# Autodesk Inventor assembly: Montiert
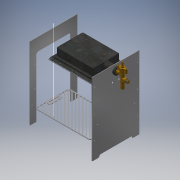
[picture p0: Inventor's stored thumbnail of the model, 180x180]
Saved by Autodesk Inventor 2018 (Build 220112000, 112)
## iProperties
Created: 2017-11-12
Part Number: Montiert
Material: Generisch
Document SubType Name: Assembly
Mass: 12109.4 g
Surface Area: 4943.53 cm^2
Volume: 1535.77 cm^3
Density: 7.8849 g/cm^3
## Documents named in this file (18)
- C:\git\RoKu-ProjectX01\Konstruktion\Montiert.iam
- C:\git\RoKu-ProjectX01\Konstruktion\Brenner.ipt
- C:\git\RoKu-ProjectX01\Konstruktion\BrennerHalter.ipt
- C:\git\RoKu-ProjectX01\Konstruktion\Gegenhalter.ipt
- C:\Users\kuckal\Documents\Inventor\Content Center Files\R2018\de-DE\ISO 7380-1\ISO 7380-1 - M4 x 6.ipt
- C:\Users\kuckal\Documents\Inventor\Content Center Files\R2018\de-DE\ISO 7380-1\ISO 7380-1 - M4 x 8.ipt
- C:\Users\kuckal\Documents\Inventor\Content Center Files\R2018\de-DE\ISO 4036(1)\ISO 4036 - M4(1).ipt
- C:\git\RoKu-ProjectX01\Konstruktion\Front.ipt
- C:\git\RoKu-ProjectX01\Konstruktion\MutterMitUScheibe.ipt
- C:\git\RoKu-ProjectX01\Konstruktion\SeiteRechts.ipt
- C:\git\RoKu-ProjectX01\Konstruktion\SeiteLinks.ipt
- C:\git\RoKu-ProjectX01\Konstruktion\Deckel.ipt
- C:\git\RoKu-ProjectX01\Konstruktion\Boden.ipt
- C:\git\RoKu-ProjectX01\Konstruktion\Back.ipt
- C:\git\RoKu-ProjectX01\Konstruktion\Gasanschluss.ipt
- C:\Users\kuckal\Documents\Inventor\Content Center Files\R2018\de-DE\DIN EN 24 036(2)\DIN EN 24 036 - M4.ipt
- C:\git\RoKu-ProjectX01\Konstruktion\EinschubRechts.ipt
- C:\git\RoKu-ProjectX01\Konstruktion\Rost_Beef.ipt
## Components (90 placed, 16 different names)
1. Brenner:1 — Fluchtend:1, Fluchtend:2, Fluchtend:3, Passend:1, Einfügen:1, Einfügen:2, Einfügen:3, Einfügen:4, Einfügen:5, Einfügen:6, Einfügen:7, Einfügen:8, Einfügen:9, Einfügen:10, Einfügen:11, Einfügen:12, Fluchtend:6, Passend:41, Passend:42
2. BrennerHalter:1 — Passend:1, Passend:2, Passend:3, Fluchtend:4, Passend:17, Fluchtend:6, Passend:18, Passend:22
3. Gegenhalter:1 — Passend:3, Passend:4, Einfügen:13, Einfügen:14, Einfügen:15, Einfügen:16, Einfügen:17, Einfügen:18, Einfügen:19, Einfügen:20, Einfügen:21, Einfügen:22, Einfügen:23, Einfügen:24
4. Front:1 — Fluchtend:4, Passend:7, Passend:8, Passend:9, Passend:10, Passend:11, Passend:12, Passend:13, Passend:14, Passend:15, Einfügen:25, Einfügen:26, Einfügen:27, Einfügen:28, Passend:16, Fluchtend:5, Passend:17, Passend:19, Fluchtend:7, Passend:21, Einfügen:37, Einfügen:38, Einfügen:39, Einfügen:40, Einfügen:41, Einfügen:42, Fluchtend:12, Fluchtend:13
5. SeiteRechts:1 — Passend:16, Fluchtend:5, Passend:18, Passend:28, Passend:29, Passend:30, Passend:31, Einfügen:29, Einfügen:30, Fluchtend:9, Fluchtend:10, Einfügen:55, Einfügen:56, Einfügen:57, Einfügen:58, Einfügen:59, Einfügen:60
6. SeiteLinks:1 — Passend:19, Fluchtend:7, Passend:20, Passend:22, Passend:24, Passend:25, Passend:26, Passend:27, Einfügen:31, Einfügen:32, Einfügen:43, Einfügen:44, Einfügen:45, Einfügen:52, Einfügen:53, Einfügen:54
7. Deckel:1 — Passend:20, Passend:21, Passend:23, Einfügen:61, Einfügen:62, Einfügen:63, Einfügen:64, Einfügen:65, Einfügen:66
8. Boden:1 — Fluchtend:8, Passend:32
9. Back:1 — Fluchtend:9, Fluchtend:10, Passend:33, Passend:34, Passend:35, Passend:36, Passend:37, Passend:38, Passend:39, Passend:40, Einfügen:33, Einfügen:34, Einfügen:35, Einfügen:36, Einfügen:46, Einfügen:47, Einfügen:48, Einfügen:49, Einfügen:50, Einfügen:51, Passend:45
10. Gasanschluss:1 — Passend:41, Passend:42, Fluchtend:11
11. EinschubRechts:1 — Fluchtend:14, Passend:43, Passend:44
12. Rost_Beef:1 — Passend:43, Passend:44, Passend:45
13. ISO 7380-1 M4 x 6:6 — Einfügen:66
14. ISO 7380-1 M4 x 6:5 — Einfügen:65
15. ISO 7380-1 M4 x 6:4 — Einfügen:64
16. ISO 7380-1 M4 x 6:3 — Einfügen:63
17. ISO 7380-1 M4 x 6:2 — Einfügen:62
18. ISO 7380-1 M4 x 6:1 — Einfügen:61
19. DIN EN 24036 M4:24 — Einfügen:60
20. DIN EN 24036 M4:23 — Einfügen:59
21. DIN EN 24036 M4:22 — Einfügen:58
22. DIN EN 24036 M4:21 — Einfügen:57
23. DIN EN 24036 M4:20 — Einfügen:56
24. DIN EN 24036 M4:19 — Einfügen:55
25. DIN EN 24036 M4:18 — Einfügen:54
26. DIN EN 24036 M4:17 — Einfügen:53
27. DIN EN 24036 M4:16 — Einfügen:52
28. ISO 7380-1 M4 x 8:36 — Einfügen:51
29. ISO 7380-1 M4 x 8:35 — Einfügen:50
30. ISO 7380-1 M4 x 8:34 — Einfügen:49
31. ISO 7380-1 M4 x 8:33 — Einfügen:48
32. ISO 7380-1 M4 x 8:32 — Einfügen:47
33. ISO 7380-1 M4 x 8:31 — Einfügen:46
34. DIN EN 24036 M4:15 — Einfügen:45
35. DIN EN 24036 M4:14 — Einfügen:44
36. DIN EN 24036 M4:13 — Einfügen:43
37. ISO 7380-1 M4 x 8:30 — Einfügen:42
38. ISO 7380-1 M4 x 8:29 — Einfügen:41
39. ISO 7380-1 M4 x 8:28 — Einfügen:40
40. ISO 7380-1 M4 x 8:27 — Einfügen:39
41. ISO 7380-1 M4 x 8:26 — Einfügen:38
42. ISO 7380-1 M4 x 8:25 — Einfügen:37
43. ISO 7380-1 M4 x 8:1 — Einfügen:1, Passend:4
44. ISO 7380-1 M4 x 8:2 — Einfügen:2
45. ISO 7380-1 M4 x 8:3 — Einfügen:3
46. ISO 7380-1 M4 x 8:4 — Einfügen:4
47. ISO 7380-1 M4 x 8:5 — Einfügen:5
48. ISO 7380-1 M4 x 8:6 — Einfügen:6
49. ISO 7380-1 M4 x 8:7 — Einfügen:7
50. ISO 7380-1 M4 x 8:8 — Einfügen:8
51. ISO 7380-1 M4 x 8:9 — Einfügen:9
52. ISO 7380-1 M4 x 8:10 — Einfügen:10
53. ISO 7380-1 M4 x 8:11 — Einfügen:11
54. ISO 7380-1 M4 x 8:12 — Einfügen:12
55. DIN EN 24036 M4:1 — Einfügen:13
56. DIN EN 24036 M4:2 — Einfügen:14
57. DIN EN 24036 M4:3 — Einfügen:15
58. DIN EN 24036 M4:4 — Einfügen:16
59. DIN EN 24036 M4:5 — Einfügen:17
60. DIN EN 24036 M4:6 — Einfügen:18
61. DIN EN 24036 M4:7 — Einfügen:19
62. DIN EN 24036 M4:8 — Einfügen:20
63. DIN EN 24036 M4:9 — Einfügen:21
64. DIN EN 24036 M4:10 — Einfügen:22
65. DIN EN 24036 M4:11 — Einfügen:23
66. DIN EN 24036 M4:12 — Einfügen:24
67. MutterMitUScheibe:9 — Passend:37, Passend:38
68. MutterMitUScheibe:10 — Passend:39, Passend:40
69. MutterMitUScheibe:11 — Passend:35, Passend:36
70. MutterMitUScheibe:12 — Passend:33, Passend:34
71. ISO 7380-1 M4 x 8:21 — Einfügen:33
72. ISO 7380-1 M4 x 8:22 — Einfügen:34
73. ISO 7380-1 M4 x 8:23 — Einfügen:35
74. ISO 7380-1 M4 x 8:24 — Einfügen:36
75. MutterMitUScheibe:5 — Passend:24, Passend:25
76. MutterMitUScheibe:6 — Passend:26, Passend:27, Passend:32
77. MutterMitUScheibe:7 — Passend:30, Passend:31
78. MutterMitUScheibe:8 — Passend:28, Passend:29
79. ISO 7380-1 M4 x 8:17 — Einfügen:29
80. ISO 7380-1 M4 x 8:18 — Einfügen:30
81. ISO 7380-1 M4 x 8:19 — Einfügen:31
82. ISO 7380-1 M4 x 8:20 — Einfügen:32
83. MutterMitUScheibe:1 — Passend:9, Passend:14
84. MutterMitUScheibe:2 — Passend:8, Passend:15
85. MutterMitUScheibe:3 — Passend:11, Passend:12
86. MutterMitUScheibe:4 — Passend:10, Passend:13
87. ISO 7380-1 M4 x 8:13 — Einfügen:25
88. ISO 7380-1 M4 x 8:14 — Einfügen:26
89. ISO 7380-1 M4 x 8:15 — Einfügen:27
90. ISO 7380-1 M4 x 8:16 — Einfügen:28
## Relationships (123: Insert 66, Mate 43, Flush 14)
- Fluchtend:1 [Flush]: Brenner:1
- Fluchtend:2 [Flush]: Brenner:1
- Fluchtend:3 [Flush]: Brenner:1
- Passend:1 [Mate]: Brenner:1 ↔ BrennerHalter:1
- Passend:2 [Mate]: BrennerHalter:1
- Passend:3 [Mate]: BrennerHalter:1 ↔ Gegenhalter:1
- Einfügen:1 [Insert]: Brenner:1 ↔ ISO 7380-1 M4 x 8:1
- Einfügen:2 [Insert]: Brenner:1 ↔ ISO 7380-1 M4 x 8:2
- Einfügen:3 [Insert]: Brenner:1 ↔ ISO 7380-1 M4 x 8:3
- Einfügen:4 [Insert]: Brenner:1 ↔ ISO 7380-1 M4 x 8:4
- Einfügen:5 [Insert]: Brenner:1 ↔ ISO 7380-1 M4 x 8:5
- Einfügen:6 [Insert]: Brenner:1 ↔ ISO 7380-1 M4 x 8:6
- Einfügen:7 [Insert]: Brenner:1 ↔ ISO 7380-1 M4 x 8:7
- Einfügen:8 [Insert]: Brenner:1 ↔ ISO 7380-1 M4 x 8:8
- Einfügen:9 [Insert]: Brenner:1 ↔ ISO 7380-1 M4 x 8:9
- Einfügen:10 [Insert]: Brenner:1 ↔ ISO 7380-1 M4 x 8:10
- Einfügen:11 [Insert]: Brenner:1 ↔ ISO 7380-1 M4 x 8:11
- Einfügen:12 [Insert]: Brenner:1 ↔ ISO 7380-1 M4 x 8:12
- Passend:4 [Mate]: Gegenhalter:1 ↔ ISO 7380-1 M4 x 8:1
- Einfügen:13 [Insert]: Gegenhalter:1 ↔ DIN EN 24036 M4:1
- Einfügen:14 [Insert]: Gegenhalter:1 ↔ DIN EN 24036 M4:2
- Einfügen:15 [Insert]: Gegenhalter:1 ↔ DIN EN 24036 M4:3
- Einfügen:16 [Insert]: Gegenhalter:1 ↔ DIN EN 24036 M4:4
- Einfügen:17 [Insert]: Gegenhalter:1 ↔ DIN EN 24036 M4:5
- Einfügen:18 [Insert]: Gegenhalter:1 ↔ DIN EN 24036 M4:6
- Einfügen:19 [Insert]: Gegenhalter:1 ↔ DIN EN 24036 M4:7
- Einfügen:20 [Insert]: Gegenhalter:1 ↔ DIN EN 24036 M4:8
- Einfügen:21 [Insert]: Gegenhalter:1 ↔ DIN EN 24036 M4:9
- Einfügen:22 [Insert]: Gegenhalter:1 ↔ DIN EN 24036 M4:10
- Einfügen:23 [Insert]: Gegenhalter:1 ↔ DIN EN 24036 M4:11
- Einfügen:24 [Insert]: Gegenhalter:1 ↔ DIN EN 24036 M4:12
- Fluchtend:4 [Flush]: BrennerHalter:1 ↔ Front:1
- Passend:7 [Mate]: Front:1
- Passend:8 [Mate]: Front:1 ↔ MutterMitUScheibe:2
- Passend:9 [Mate]: Front:1 ↔ MutterMitUScheibe:1
- Passend:10 [Mate]: Front:1 ↔ MutterMitUScheibe:4
- Passend:11 [Mate]: Front:1 ↔ MutterMitUScheibe:3
- Passend:12 [Mate]: Front:1 ↔ MutterMitUScheibe:3
- Passend:13 [Mate]: Front:1 ↔ MutterMitUScheibe:4
- Passend:14 [Mate]: Front:1 ↔ MutterMitUScheibe:1
- Passend:15 [Mate]: Front:1 ↔ MutterMitUScheibe:2
- Einfügen:25 [Insert]: Front:1 ↔ ISO 7380-1 M4 x 8:13
- Einfügen:26 [Insert]: Front:1 ↔ ISO 7380-1 M4 x 8:14
- Einfügen:27 [Insert]: Front:1 ↔ ISO 7380-1 M4 x 8:15
- Einfügen:28 [Insert]: Front:1 ↔ ISO 7380-1 M4 x 8:16
- Passend:16 [Mate]: Front:1 ↔ SeiteRechts:1
- Fluchtend:5 [Flush]: Front:1 ↔ SeiteRechts:1
- Passend:17 [Mate]: BrennerHalter:1 ↔ Front:1
- Fluchtend:6 [Flush] (-10 mm): Brenner:1 ↔ BrennerHalter:1
- Passend:18 [Mate]: BrennerHalter:1 ↔ SeiteRechts:1
- Passend:19 [Mate]: Front:1 ↔ SeiteLinks:1
- Fluchtend:7 [Flush]: Front:1 ↔ SeiteLinks:1
- Passend:20 [Mate]: SeiteLinks:1 ↔ Deckel:1
- Passend:21 [Mate]: Front:1 ↔ Deckel:1
- Passend:22 [Mate]: BrennerHalter:1 ↔ SeiteLinks:1
- Passend:23 [Mate]: Deckel:1
- Passend:24 [Mate]: SeiteLinks:1 ↔ MutterMitUScheibe:5
- Passend:25 [Mate]: SeiteLinks:1 ↔ MutterMitUScheibe:5
- Passend:26 [Mate]: SeiteLinks:1 ↔ MutterMitUScheibe:6
- Passend:27 [Mate]: SeiteLinks:1 ↔ MutterMitUScheibe:6
- Passend:28 [Mate]: SeiteRechts:1 ↔ MutterMitUScheibe:8
- Passend:29 [Mate]: SeiteRechts:1 ↔ MutterMitUScheibe:8
- Passend:30 [Mate]: SeiteRechts:1 ↔ MutterMitUScheibe:7
- Passend:31 [Mate]: SeiteRechts:1 ↔ MutterMitUScheibe:7
- Einfügen:29 [Insert]: SeiteRechts:1 ↔ ISO 7380-1 M4 x 8:17
- Einfügen:30 [Insert]: SeiteRechts:1 ↔ ISO 7380-1 M4 x 8:18
- Einfügen:31 [Insert]: SeiteLinks:1 ↔ ISO 7380-1 M4 x 8:19
- Einfügen:32 [Insert]: SeiteLinks:1 ↔ ISO 7380-1 M4 x 8:20
- Fluchtend:8 [Flush]: Boden:1
- Passend:32 [Mate]: Boden:1 ↔ MutterMitUScheibe:6
- Fluchtend:9 [Flush]: SeiteRechts:1 ↔ Back:1
- Fluchtend:10 [Flush]: SeiteRechts:1 ↔ Back:1
- Passend:33 [Mate]: Back:1 ↔ MutterMitUScheibe:12
- Passend:34 [Mate]: Back:1 ↔ MutterMitUScheibe:12
- Passend:35 [Mate]: Back:1 ↔ MutterMitUScheibe:11
- Passend:36 [Mate]: Back:1 ↔ MutterMitUScheibe:11
- Passend:37 [Mate]: Back:1 ↔ MutterMitUScheibe:9
- Passend:38 [Mate]: Back:1 ↔ MutterMitUScheibe:9
- Passend:39 [Mate]: Back:1 ↔ MutterMitUScheibe:10
- Passend:40 [Mate]: Back:1 ↔ MutterMitUScheibe:10
- Einfügen:33 [Insert]: Back:1 ↔ ISO 7380-1 M4 x 8:21
- Einfügen:34 [Insert]: Back:1 ↔ ISO 7380-1 M4 x 8:22
- Einfügen:35 [Insert]: Back:1 ↔ ISO 7380-1 M4 x 8:23
- Einfügen:36 [Insert]: Back:1 ↔ ISO 7380-1 M4 x 8:24
- Passend:41 [Mate]: Brenner:1 ↔ Gasanschluss:1
- Passend:42 [Mate]: Brenner:1 ↔ Gasanschluss:1
- Fluchtend:11 [Flush]: Gasanschluss:1
- Einfügen:37 [Insert]: Front:1 ↔ ISO 7380-1 M4 x 8:25
- Einfügen:38 [Insert]: Front:1 ↔ ISO 7380-1 M4 x 8:26
- Einfügen:39 [Insert]: Front:1 ↔ ISO 7380-1 M4 x 8:27
- Einfügen:40 [Insert]: Front:1 ↔ ISO 7380-1 M4 x 8:28
- Einfügen:41 [Insert]: Front:1 ↔ ISO 7380-1 M4 x 8:29
- Einfügen:42 [Insert]: Front:1 ↔ ISO 7380-1 M4 x 8:30
- Einfügen:43 [Insert]: SeiteLinks:1 ↔ DIN EN 24036 M4:13
- Einfügen:44 [Insert]: SeiteLinks:1 ↔ DIN EN 24036 M4:14
- Einfügen:45 [Insert]: SeiteLinks:1 ↔ DIN EN 24036 M4:15
- Einfügen:46 [Insert]: Back:1 ↔ ISO 7380-1 M4 x 8:31
- Einfügen:47 [Insert]: Back:1 ↔ ISO 7380-1 M4 x 8:32
- Einfügen:48 [Insert]: Back:1 ↔ ISO 7380-1 M4 x 8:33
- Einfügen:49 [Insert]: Back:1 ↔ ISO 7380-1 M4 x 8:34
- Einfügen:50 [Insert]: Back:1 ↔ ISO 7380-1 M4 x 8:35
- Einfügen:51 [Insert]: Back:1 ↔ ISO 7380-1 M4 x 8:36
- Einfügen:52 [Insert]: SeiteLinks:1 ↔ DIN EN 24036 M4:16
- Einfügen:53 [Insert]: SeiteLinks:1 ↔ DIN EN 24036 M4:17
- Einfügen:54 [Insert]: SeiteLinks:1 ↔ DIN EN 24036 M4:18
- Einfügen:55 [Insert]: SeiteRechts:1 ↔ DIN EN 24036 M4:19
- Einfügen:56 [Insert]: SeiteRechts:1 ↔ DIN EN 24036 M4:20
- Einfügen:57 [Insert]: SeiteRechts:1 ↔ DIN EN 24036 M4:21
- Einfügen:58 [Insert]: SeiteRechts:1 ↔ DIN EN 24036 M4:22
- Einfügen:59 [Insert]: SeiteRechts:1 ↔ DIN EN 24036 M4:23
- Einfügen:60 [Insert]: SeiteRechts:1 ↔ DIN EN 24036 M4:24
- Einfügen:61 [Insert]: Deckel:1 ↔ ISO 7380-1 M4 x 6:1
- Einfügen:62 [Insert]: Deckel:1 ↔ ISO 7380-1 M4 x 6:2
- Einfügen:63 [Insert]: Deckel:1 ↔ ISO 7380-1 M4 x 6:3
- Einfügen:64 [Insert]: Deckel:1 ↔ ISO 7380-1 M4 x 6:4
- Einfügen:65 [Insert]: Deckel:1 ↔ ISO 7380-1 M4 x 6:5
- Einfügen:66 [Insert]: Deckel:1 ↔ ISO 7380-1 M4 x 6:6
- Fluchtend:12 [Flush] (3 mm): Front:1
- Fluchtend:13 [Flush] (5 mm): Front:1
- Fluchtend:14 [Flush]: EinschubRechts:1
- Passend:43 [Mate]: EinschubRechts:1 ↔ Rost_Beef:1
- Passend:44 [Mate] (0.125 mm): EinschubRechts:1 ↔ Rost_Beef:1
- Passend:45 [Mate] (38 mm): Back:1 ↔ Rost_Beef:1
